# Autodesk Inventor assembly: axis5_6 smaller v1
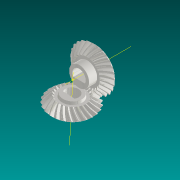
[picture p0: Inventor's stored thumbnail of the model, 180x180]
Saved by Autodesk Inventor 2020.3 (Build 243373000, 373)
## iProperties
Created: 2020-05-25
Part Number: axis5_6 smaller v1
Document SubType Name: Assembly
Designer: stefa
Author: stefa
## Documents named in this file (2)
- C:\Users\Svend\OneDrive\Documents\GitHub\BeerMinder\3D-model\axis5_6\tandwiel assemble.iam
- C:\Users\Svend\OneDrive\Documents\GitHub\BeerMinder\3D-model\axis5_6\axis5_6 smaller v1\Design Accelerator\Bevel Gears1.iam
## Components (1 placed, 1 different names)
1. Bevel Gears assemble:1 [sub-assembly] — Mate:1, Mate:2
## Relationships (2: Mate 2)
- Mate:1: Bevel Gears assemble:1
- Mate:2: Bevel Gears assemble:1
